# Autodesk Inventor assembly: Moving Carousel Single
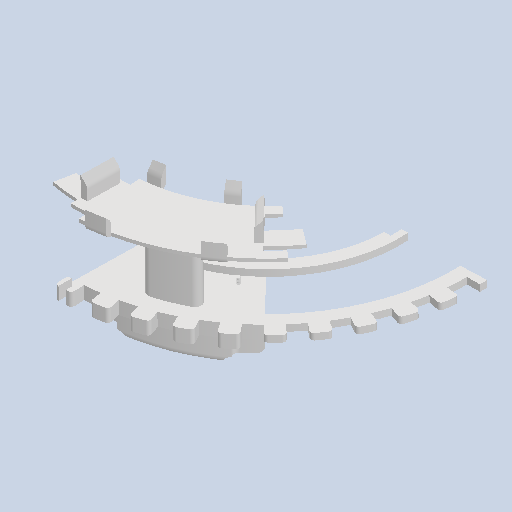
[picture p0: Inventor's stored thumbnail of the model, 512x512]
Saved by Autodesk Inventor 2023 (Build 270158000, 158)
## iProperties
Created: 2023-01-28
Part Number: Moving Carousel Single
Document SubType Name: Assembly
Designer: cheng
Author: cheng
## Documents named in this file (3)
- C:\Users\cheng\Desktop\4th Year Project\Inventor\Ninth Assembly\Moving Carousel Single.iam
- C:\Users\cheng\Desktop\4th Year Project\Inventor\Ninth Assembly\Moving Carousel V3.ipt
- C:\Users\cheng\Desktop\4th Year Project\Inventor\Ninth Assembly\WDS568-219-STEP-AP203\WDS568-219.ipt
## Components (3 placed, 2 different names)
1. Moving Carousel V3:1 — Mate:1, Mate:2, Mate:4, Mate:5
2. WDS568-219:2 — Mate:2, Mate:5
3. WDS568-219:3 — Mate:1, Mate:4
## Relationships (4: Mate 4)
- Mate:1: Moving Carousel V3:1 ↔ WDS568-219:3
- Mate:2: Moving Carousel V3:1 ↔ WDS568-219:2
- Mate:4: Moving Carousel V3:1 ↔ WDS568-219:3
- Mate:5: Moving Carousel V3:1 ↔ WDS568-219:2
